# Autodesk Inventor assembly: pendulum_assembly
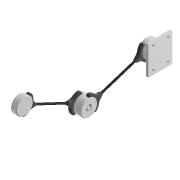
[picture p0: Inventor's stored thumbnail of the model, 180x180]
Saved by Autodesk Inventor 2017 (Build 210142000, 142)
## iProperties
Created: 2017-12-13
Part Number: pendulum_assembly
Document SubType Name: Assembly
Designer: Thoma
Author: Thoma
## Documents named in this file (7)
- C:\Users\Thoma\Documents\SDUEmbedded\pendulum\joint\pendulum_assembly.iam
- C:\Users\Thoma\Documents\SDUEmbedded\pendulum\joint\joint_assembly.iam
- C:\Users\Thoma\Documents\master\components\joint\joint_mount.ipt
- C:\Users\Thoma\Documents\master\components\joint\mounting_plate.ipt
- C:\Users\Thoma\Documents\SDUEmbedded\pendulum\joint\joint_mag_assembly.iam
- C:\Users\Thoma\Documents\SDUEmbedded\pendulum\joint\dummy_disc.ipt
- C:\Users\Thoma\Documents\SDUEmbedded\pendulum\joint\carbon_rod.ipt
## Components (12 placed, 6 different names)
1. joint_assembly:1 [sub-assembly] — Mate:9, Mate:10, Angle:1, Mate:27, Mate:28
2. joint_mount:1 — Mate:19, Mate:21, Mate:22, Mate:24, Mate:27, Mate:28
3. mounting_plate:1 — Mate:3, Mate:4, Mate:5, Mate:6, Mate:7, Mate:8
4. joint_mag_assembly:1 [sub-assembly] — Mate:6, Mate:7, Mate:8, Mate:9, Mate:10
5. joint_assembly:2 [sub-assembly] — Mate:11, Mate:12, Angle:1, Angle:2, Mate:29, Mate:30
6. joint_mag_assembly:2 [sub-assembly] — Mate:11, Mate:12, Mate:15, Mate:16
7. dummy_disc:1 — Mate:17, Mate:18, Angle:2
8. joint_mount:2 — Mate:20, Mate:23, Mate:25, Mate:26, Mate:29, Mate:30
9. joint_mount:3 — Mate:17, Mate:18, Mate:20, Mate:26
10. joint_mount:4 — Mate:15, Mate:16, Mate:19, Mate:22
11. carbon_rod:1 — Mate:21, Mate:24
12. carbon_rod:2 — Mate:23, Mate:25
## Relationships (28: Mate 26, Angle 2)
- Mate:3: mounting_plate:1
- Mate:4: mounting_plate:1
- Mate:5: mounting_plate:1
- Mate:6: mounting_plate:1 ↔ joint_mag_assembly:1
- Mate:7: mounting_plate:1 ↔ joint_mag_assembly:1
- Mate:8: mounting_plate:1 ↔ joint_mag_assembly:1
- Mate:9: joint_assembly:1 ↔ joint_mag_assembly:1
- Mate:10 (1 mm): joint_assembly:1 ↔ joint_mag_assembly:1
- Mate:11: joint_assembly:2 ↔ joint_mag_assembly:2
- Mate:12 (1 mm): joint_assembly:2 ↔ joint_mag_assembly:2
- Mate:15: joint_mag_assembly:2 ↔ joint_mount:4
- Mate:16: joint_mag_assembly:2 ↔ joint_mount:4
- Mate:17: dummy_disc:1 ↔ joint_mount:3
- Mate:18: dummy_disc:1 ↔ joint_mount:3
- Mate:19: joint_mount:1 ↔ joint_mount:4
- Mate:20: joint_mount:2 ↔ joint_mount:3
- Angle:1 (0 deg): joint_assembly:1 ↔ joint_assembly:2
- Angle:2 (0 deg): joint_assembly:2 ↔ dummy_disc:1
- Mate:21: joint_mount:1 ↔ carbon_rod:1
- Mate:22 (150 mm): joint_mount:1 ↔ joint_mount:4
- Mate:23: joint_mount:2 ↔ carbon_rod:2
- Mate:24 (-20 mm): joint_mount:1 ↔ carbon_rod:1
- Mate:25 (-20 mm): joint_mount:2 ↔ carbon_rod:2
- Mate:26 (150 mm): joint_mount:2 ↔ joint_mount:3
- Mate:27: joint_assembly:1 ↔ joint_mount:1
- Mate:28: joint_assembly:1 ↔ joint_mount:1
- Mate:29: joint_assembly:2 ↔ joint_mount:2
- Mate:30: joint_assembly:2 ↔ joint_mount:2
